# Autodesk Inventor assembly: Rendering
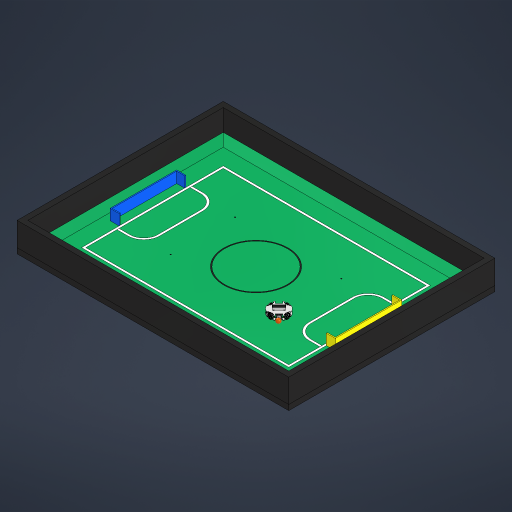
[picture p0: Inventor's stored thumbnail of the model, 512x512]
Saved by Autodesk Inventor 2024.2 (Build 282272000, 272)
## iProperties
Created: 2023-12-22
Part Number: Rendering
Document SubType Name: Assembly
Designer: Hanaoka
Author: Hanaoka
## Documents named in this file (3)
- G:\共有ドライブ\reRo\05_個人\hanaoka\inventor\Field\Rendering.iam
- G:\共有ドライブ\reRo\05_個人\hanaoka\inventor\Field\Field_2020\Field_2020.ipt
- G:\共有ドライブ\reRo\05_個人\hanaoka\inventor\Attacker_v1.iam
## Components (2 placed, 2 different names)
1. Field_2020:1 — メイト:1, メイト:2
2. Attacker_v1:1 [sub-assembly]
## Relationships (2: Mate 2)
- メイト:1 [Mate]: Field_2020:1
- メイト:2 [Mate] (-960 mm): Field_2020:1
